# Autodesk Inventor assembly: surround_assembly
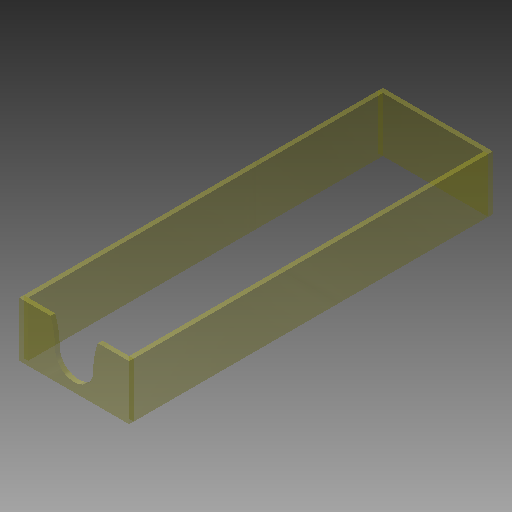
[picture p0: Inventor's stored thumbnail of the model, 512x512]
Saved by Autodesk Inventor 2018.1 (Build 221171000, 171)
## iProperties
Created: 2017-07-30
Part Number: surround_assembly
Document SubType Name: Assembly
Designer: Tom
Author: Tom
## Documents named in this file (4)
- \\Mac\Dropbox\2015-2016\Bachelorproef\Inventor\Etstank_v2\surround_assembly.iam
- \\Mac\Dropbox\2015-2016\Bachelorproef\Inventor\Etstank_v2\surround_side.ipt
- \\Mac\Dropbox\2015-2016\Bachelorproef\Inventor\Etstank_v2\surround_front.ipt
- \\Mac\Dropbox\2015-2016\Bachelorproef\Inventor\Etstank_v2\surround_back.ipt
## Components (4 placed, 3 different names)
1. surround_side:1 — Mate:2, Flush:1, Flush:4
2. surround_side:2 — Mate:1, Flush:2, Flush:3, Mate:3, Flush:5, Flush:6
3. surround_front:1 — Mate:1, Mate:2, Flush:1, Flush:2, Flush:3, Flush:4
4. surround_back:1 — Mate:3, Flush:5, Flush:6
## Relationships (9: Flush 6, Mate 3)
- Mate:1: surround_side:2 ↔ surround_front:1
- Mate:2: surround_side:1 ↔ surround_front:1
- Flush:1: surround_side:1 ↔ surround_front:1
- Flush:2: surround_side:2 ↔ surround_front:1
- Flush:3: surround_side:2 ↔ surround_front:1
- Flush:4: surround_side:1 ↔ surround_front:1
- Mate:3: surround_side:2 ↔ surround_back:1
- Flush:5: surround_side:2 ↔ surround_back:1
- Flush:6: surround_side:2 ↔ surround_back:1
